# Autodesk Inventor assembly: Large_drone_assembly_V2
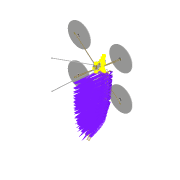
[picture p0: Inventor's stored thumbnail of the model, 180x180]
Saved by Autodesk Inventor 2022 (Build 260153000, 153)
## iProperties
Created: 2022-04-28
Part Number: Large_drone_assembly_V2
Document SubType Name: Assembly
Designer: dell
Mass: 4396.41 g
Surface Area: 10173.4 cm^2
Volume: 3712.61 cm^3
Density: 1.18418 g/cm^3
Author: dell
## Documents named in this file (13)
- D:\xxxx\Uni\Part IV\MECHENG_700\Part_IV_project_CAD\Bird_skeleton_prototypes\Wing_drone_V1\Large_drone_assembly_V2.iam
- D:\xxxx\Uni\Part IV\MECHENG_700\Part_IV_project_CAD\Bird_skeleton_prototypes\Wing_drone_V1\Drone_plate_1.ipt
- D:\xxxx\Uni\Part IV\MECHENG_700\Part_IV_project_CAD\Bird_skeleton_prototypes\Wing_drone_V1\Blade_simulator.ipt
- D:\xxxx\Uni\Part IV\MECHENG_700\Part_IV_project_CAD\Bird_skeleton_prototypes\Wing_drone_V1\Landing_leg\Landing_leg_assembly.iam
- D:\xxxx\Uni\Part IV\MECHENG_700\Part_IV_project_CAD\Bird_skeleton_prototypes\Wing_drone_V1\M3_spacer_27mm.ipt
- D:\xxxx\Uni\Part IV\MECHENG_700\Part_IV_project_CAD\Bird_skeleton_prototypes\Wing_drone_V1\Drone_plate_3.ipt
- D:\xxxx\Uni\Part IV\MECHENG_700\Part_IV_project_CAD\Bird_skeleton_prototypes\Wing_drone_V1\Foam_wing\Foam_wing.iam
- D:\xxxx\Uni\Part IV\MECHENG_700\Part_IV_project_CAD\Bird_skeleton_prototypes\Wing_drone_V1\Bird_wing_V2\Wing_shoulder\Shoulder_support_assembly.iam
- D:\xxxx\Uni\Part IV\MECHENG_700\Part_IV_project_CAD\Bird_skeleton_prototypes\Wing_drone_V1\Large_drone_rotor_arm_assembly.iam
- D:\xxxx\Uni\Part IV\MECHENG_700\Part_IV_project_CAD\Bird_skeleton_prototypes\Wing_drone_V1\Electronics\Electronics_assembly.iam
- D:\xxxx\Uni\Part IV\MECHENG_700\Part_IV_project_CAD\Bird_skeleton_prototypes\Wing_drone_V1\Electronics\Pixhawk4.ipt
- D:\xxxx\Uni\Part IV\MECHENG_700\Part_IV_project_CAD\Bird_skeleton_prototypes\Wing_drone_V1\Bird_wing_V2\Bird_wing_assembly_V2.iam
- D:\xxxx\Uni\Part IV\MECHENG_700\Part_IV_project_CAD\Bird_skeleton_prototypes\Wing_drone_V1\Bird_wing_V2\Primary_hinge_guide_pulley.ipt
## Components (25 placed, 12 different names)
1. Drone_plate_1:1 — Flush:1, Flush:2, Mate:65, Mate:66, Mate:67, Mate:79, Mate:80, Mate:81, Mate:82, Mate:83, Mate:84, Mate:85, Mate:86, Mate:87, Mate:90, Mate:100, Mate:106, Mate:107, Mate:108, Mate:111, Mate:112, Mate:113, Mate:116, Mate:117, Mate:118, Mate:121, Mate:122, Mate:123
2. Blade_simulator:1 — Mate:109, Mate:110
3. Blade_simulator:2 — Mate:124, Mate:125
4. Blade_simulator:3 — Mate:114, Mate:115
5. Blade_simulator:4 — Mate:119, Mate:120
6. Drone_plate_1:2 — Flush:1, Flush:2, Mate:69, Mate:71, Mate:72, Mate:73, Mate:74, Mate:75, Mate:88, Mate:89, Mate:98, Mate:99, Mate:130
7. Landing_leg_assembly:1 [sub-assembly] — Mate:65, Mate:66, Mate:67
8. M3_spacer_27mm:1 — Mate:69, Mate:127
9. M3_spacer_27mm:2 — Mate:71, Mate:126
10. M3_spacer_27mm:3 — Mate:72, Mate:73, Mate:76
11. M3_spacer_27mm:4 — Mate:74, Mate:75, Mate:77, Mate:78
12. Drone_plate_3:1 — Mate:76, Mate:77, Mate:78, Mate:126, Mate:127, Mate:132, Mate:133, Mate:134, Mate:135
13. Landing_leg_assembly:2 [sub-assembly] — Mate:85, Mate:86, Mate:87
14. Landing_leg_assembly:3 [sub-assembly] — Mate:82, Mate:83, Mate:84
15. Landing_leg_assembly:4 [sub-assembly] — Mate:79, Mate:80, Mate:81
16. Foam_wing:1 [sub-assembly] — Mate:88, Mate:89, Mate:90
17. Shoulder_support_assembly:1 [sub-assembly] — Mate:98, Mate:99, Mate:100, Mate:136, Mate:137, Mate:139, Mate:140
18. Large_drone_rotor_arm_assembly:1 [sub-assembly] — Mate:106, Mate:107, Mate:108, Mate:109, Mate:110, Mate:130
19. Large_drone_rotor_arm_assembly:2 [sub-assembly] — Mate:111, Mate:112, Mate:113, Mate:114, Mate:115
20. Large_drone_rotor_arm_assembly:3 [sub-assembly] — Mate:116, Mate:117, Mate:118, Mate:119, Mate:120
21. Large_drone_rotor_arm_assembly:4 [sub-assembly] — Mate:121, Mate:122, Mate:123, Mate:124, Mate:125
22. Electronics_assembly:2 [sub-assembly] — Mate:133, Mate:134, Mate:135
23. Pixhawk4:2 — Mate:132
24. Bird_wing_assembly_V2:1 [sub-assembly] — Mate:136, Mate:137
25. Primary_hinge_guide_pulley:1 — Mate:139, Mate:140
## Relationships (60: Mate 58, Flush 2)
- Flush:1: Drone_plate_1:1 ↔ Drone_plate_1:2
- Flush:2: Drone_plate_1:1 ↔ Drone_plate_1:2
- Mate:65: Drone_plate_1:1 ↔ Landing_leg_assembly:1
- Mate:66: Drone_plate_1:1 ↔ Landing_leg_assembly:1
- Mate:67: Drone_plate_1:1 ↔ Landing_leg_assembly:1
- Mate:69: Drone_plate_1:2 ↔ M3_spacer_27mm:1
- Mate:71: Drone_plate_1:2 ↔ M3_spacer_27mm:2
- Mate:72: Drone_plate_1:2 ↔ M3_spacer_27mm:3
- Mate:73: Drone_plate_1:2 ↔ M3_spacer_27mm:3
- Mate:74: Drone_plate_1:2 ↔ M3_spacer_27mm:4
- Mate:75: Drone_plate_1:2 ↔ M3_spacer_27mm:4
- Mate:76: M3_spacer_27mm:3 ↔ Drone_plate_3:1
- Mate:77: M3_spacer_27mm:4 ↔ Drone_plate_3:1
- Mate:78: M3_spacer_27mm:4 ↔ Drone_plate_3:1
- Mate:79: Drone_plate_1:1 ↔ Landing_leg_assembly:4
- Mate:80: Drone_plate_1:1 ↔ Landing_leg_assembly:4
- Mate:81: Drone_plate_1:1 ↔ Landing_leg_assembly:4
- Mate:82: Drone_plate_1:1 ↔ Landing_leg_assembly:3
- Mate:83: Drone_plate_1:1 ↔ Landing_leg_assembly:3
- Mate:84: Drone_plate_1:1 ↔ Landing_leg_assembly:3
- Mate:85: Drone_plate_1:1 ↔ Landing_leg_assembly:2
- Mate:86: Drone_plate_1:1 ↔ Landing_leg_assembly:2
- Mate:87: Drone_plate_1:1 ↔ Landing_leg_assembly:2
- Mate:88: Drone_plate_1:2 ↔ Foam_wing:1
- Mate:89: Drone_plate_1:2 ↔ Foam_wing:1
- Mate:90: Drone_plate_1:1 ↔ Foam_wing:1
- Mate:98: Drone_plate_1:2 ↔ Shoulder_support_assembly:1
- Mate:99: Drone_plate_1:2 ↔ Shoulder_support_assembly:1
- Mate:100: Drone_plate_1:1 ↔ Shoulder_support_assembly:1
- Mate:106: Drone_plate_1:1 ↔ Large_drone_rotor_arm_assembly:1
- Mate:107: Drone_plate_1:1 ↔ Large_drone_rotor_arm_assembly:1
- Mate:108: Drone_plate_1:1 ↔ Large_drone_rotor_arm_assembly:1
- Mate:109: Blade_simulator:1 ↔ Large_drone_rotor_arm_assembly:1
- Mate:110: Blade_simulator:1 ↔ Large_drone_rotor_arm_assembly:1
- Mate:111: Drone_plate_1:1 ↔ Large_drone_rotor_arm_assembly:2
- Mate:112: Drone_plate_1:1 ↔ Large_drone_rotor_arm_assembly:2
- Mate:113: Drone_plate_1:1 ↔ Large_drone_rotor_arm_assembly:2
- Mate:114: Blade_simulator:3 ↔ Large_drone_rotor_arm_assembly:2
- Mate:115: Blade_simulator:3 ↔ Large_drone_rotor_arm_assembly:2
- Mate:116: Drone_plate_1:1 ↔ Large_drone_rotor_arm_assembly:3
- Mate:117: Drone_plate_1:1 ↔ Large_drone_rotor_arm_assembly:3
- Mate:118: Drone_plate_1:1 ↔ Large_drone_rotor_arm_assembly:3
- Mate:119: Blade_simulator:4 ↔ Large_drone_rotor_arm_assembly:3
- Mate:120: Blade_simulator:4 ↔ Large_drone_rotor_arm_assembly:3
- Mate:121: Drone_plate_1:1 ↔ Large_drone_rotor_arm_assembly:4
- Mate:122: Drone_plate_1:1 ↔ Large_drone_rotor_arm_assembly:4
- Mate:123: Drone_plate_1:1 ↔ Large_drone_rotor_arm_assembly:4
- Mate:124: Blade_simulator:2 ↔ Large_drone_rotor_arm_assembly:4
- Mate:125: Blade_simulator:2 ↔ Large_drone_rotor_arm_assembly:4
- Mate:126: M3_spacer_27mm:2 ↔ Drone_plate_3:1
- Mate:127: M3_spacer_27mm:1 ↔ Drone_plate_3:1
- Mate:130: Drone_plate_1:2 ↔ Large_drone_rotor_arm_assembly:1
- Mate:132: Drone_plate_3:1 ↔ Pixhawk4:2
- Mate:133: Drone_plate_3:1 ↔ Electronics_assembly:2
- Mate:134: Drone_plate_3:1 ↔ Electronics_assembly:2
- Mate:135 (0.15 mm): Drone_plate_3:1 ↔ Electronics_assembly:2
- Mate:136: Shoulder_support_assembly:1 ↔ Bird_wing_assembly_V2:1
- Mate:137: Shoulder_support_assembly:1 ↔ Bird_wing_assembly_V2:1
- Mate:139: Shoulder_support_assembly:1 ↔ Primary_hinge_guide_pulley:1
- Mate:140: Shoulder_support_assembly:1 ↔ Primary_hinge_guide_pulley:1
